# Autodesk Inventor assembly: WheelSuspension
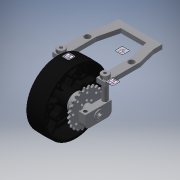
[picture p0: Inventor's stored thumbnail of the model, 180x180]
Saved by Autodesk Inventor 2017 (Build 210142000, 142)
## iProperties
Created: 2018-05-04
Part Number: WheelSuspension
Document SubType Name: Assembly
Designer: User
Author: User
## Documents named in this file (9)
- C:\Robotics\CAD\2018-19_CAD\Offseason\WheelSuspension.iam
- C:\Robotics\CAD\COTSParts\Fasteners\97345A207_316 STAINLESS STEEL SHOULDER SCREW.ipt
- C:\Robotics\CAD\COTSParts\Wheels\4in Wheel Intergreated Hub 8mm Rev2.ipt
- C:\Robotics\CAD\2016-17_CAD\Custom COTS\4inax.ipt
- C:\Robotics\CAD\2018-19_CAD\Offseason\WheelSuspensionHub.ipt
- C:\Robotics\CAD\COTSParts\Actobotics\535 parts\535198Bearing.25ID.5OD.ipt
- C:\Robotics\CAD\2018-19_CAD\Offseason\WheelandSprocketComboHub2.ipt
- C:\Robotics\CAD\COTSParts\Actobotics\615 parts\615106Sprocket.5inBore.25inPitch24Teeth.ipt
- C:\Robotics\CAD\2018-19_CAD\Offseason\WheelSuspensionFork.ipt
## Components (11 placed, 8 different names)
1. 97345A207_316 STAINLESS STEEL SHOULDER SCREW:1 — Insert:3, Mate:3, Insert:11
2. 4in Wheel Intergreated Hub 8mm Rev2:1 — Insert:6
3. 4inax:1 — Insert:2
4. WheelSuspensionHub:1 — Insert:1, Insert:3, Insert:4, Mate:2
5. 535198Bearing.25ID.5OD:1 — Insert:1, Insert:2
6. WheelandSprocketComboHub2:1 — Insert:4, Insert:5, Insert:6
7. 615106Sprocket.5inBore.25inPitch24Teeth:1 — Insert:5
8. WheelSuspensionHub:2 — Insert:7, Insert:9
9. 97345A207_316 STAINLESS STEEL SHOULDER SCREW:2 — Insert:9, Insert:10, Mate:3
10. 535198Bearing.25ID.5OD:2 — Insert:7, Mate:2
11. WheelSuspensionFork:1 — Insert:10, Insert:11, Angle:1
## Relationships (13: Insert 10, Mate 2, Angle 1)
- Insert:1: WheelSuspensionHub:1 ↔ 535198Bearing.25ID.5OD:1
- Insert:2 (3.175 mm): 4inax:1 ↔ 535198Bearing.25ID.5OD:1
- Insert:3: 97345A207_316 STAINLESS STEEL SHOULDER SCREW:1 ↔ WheelSuspensionHub:1
- Insert:4 (1.27 mm): WheelSuspensionHub:1 ↔ WheelandSprocketComboHub2:1
- Insert:5: WheelandSprocketComboHub2:1 ↔ 615106Sprocket.5inBore.25inPitch24Teeth:1
- Insert:6: 4in Wheel Intergreated Hub 8mm Rev2:1 ↔ WheelandSprocketComboHub2:1
- Insert:7: WheelSuspensionHub:2 ↔ 535198Bearing.25ID.5OD:2
- Insert:9: WheelSuspensionHub:2 ↔ 97345A207_316 STAINLESS STEEL SHOULDER SCREW:2
- Insert:10: 97345A207_316 STAINLESS STEEL SHOULDER SCREW:2 ↔ WheelSuspensionFork:1
- Mate:2: WheelSuspensionHub:1 ↔ 535198Bearing.25ID.5OD:2
- Mate:3 (63.5 mm): 97345A207_316 STAINLESS STEEL SHOULDER SCREW:1 ↔ 97345A207_316 STAINLESS STEEL SHOULDER SCREW:2
- Insert:11: 97345A207_316 STAINLESS STEEL SHOULDER SCREW:1 ↔ WheelSuspensionFork:1
- Angle:1 (0 deg): WheelSuspensionFork:1
